# Autodesk Inventor assembly: A600KBv2
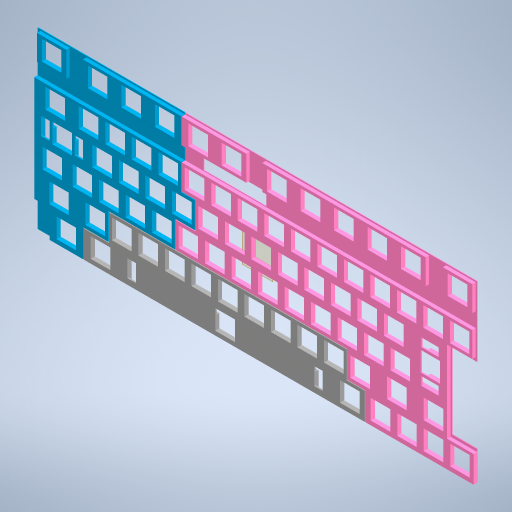
[picture p0: Inventor's stored thumbnail of the model, 512x512]
Saved by Autodesk Inventor 2024 (Build 280153000, 153)
## iProperties
Created: 2024-06-29
Part Number: A600KBv2
Document SubType Name: Assembly
Designer: adam
Author: adam
## Documents named in this file (5)
- C:\Users\adam\Projects\A600KBv2\3dprint\A600KBv2.iam
- C:\Users\adam\Projects\A600KBv2\3dprint\Plate.ipt
- C:\Users\adam\Projects\A600KBv2\3dprint\Lower Middle Plate.ipt
- C:\Users\adam\Projects\A600KBv2\3dprint\Upper Right Plate.ipt
- C:\Users\adam\Projects\A600KBv2\3dprint\Upper Left Plate.ipt
## Components (4 placed, 4 different names)
1. Plate:1 — Flush:1, Flush:2, Flush:3
2. Lower Middle Plate:1 — Flush:1
3. Upper Right Plate:1 — Flush:2
4. Upper Left Plate:1 — Flush:3
## Relationships (3: Flush 3)
- Flush:1: Plate:1 ↔ Lower Middle Plate:1
- Flush:2: Plate:1 ↔ Upper Right Plate:1
- Flush:3: Plate:1 ↔ Upper Left Plate:1
## Named parameters: plategap = 0.5 mm
